# Autodesk Inventor assembly: electronicsLayout
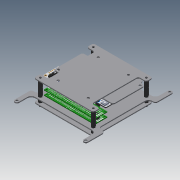
[picture p0: Inventor's stored thumbnail of the model, 180x180]
Saved by Autodesk Inventor 2018 (Build 220112000, 112)
## iProperties
Created: 2020-02-04
Part Number: electronicsLayout
Document SubType Name: Assembly
Designer: anirudh.bali
Author: anirudh.bali
## Documents named in this file (11)
- D:\Silicon Sharks\2019-2020\ElectronicsHousing\Prototype3\electronicsLayout.iam
- D:\Silicon Sharks\2019-2020\ElectronicsHousing\Prototype3\bottomPlate.ipt
- D:\Silicon Sharks\2019-2020\ElectronicsHousing\Components\standoffs\Separador plastico negro H-M M3x6x6mm.ipt
- D:\Silicon Sharks\2019-2020\ElectronicsHousing\Prototype3\groundPlate.ipt
- D:\Silicon Sharks\2019-2020\ElectronicsHousing\Components\Adafruit_BNO055_AP214.ipt
- D:\Silicon Sharks\2019-2020\ElectronicsHousing\Components\arduinoUnoDetailed.ipt
- D:\Silicon Sharks\2019-2020\ElectronicsHousing\Components\PCB2x8.ipt
- D:\Silicon Sharks\2019-2020\ElectronicsHousing\Prototype3\escPlate.ipt
- D:\Silicon Sharks\2019-2020\ElectronicsHousing\Components\standoffs\Separador plastico negro H-M M3x10x6mm.ipt
- D:\Silicon Sharks\2019-2020\ElectronicsHousing\Components\standoffs\Separador plastico negro H-M M3x12x6mm.ipt
- D:\Silicon Sharks\2019-2020\ElectronicsHousing\Prototype3\ethernetPlate.ipt
## Components (29 placed, 10 different names)
1. bottomPlate:1 — Mate:1, Mate:2, Mate:3, Mate:4, Mate:5, Mate:6, Mate:7, Mate:8
2. Separador plastico negro H-M M3x6x6mm:1 — Mate:1, Mate:5, Mate:10
3. Separador plastico negro H-M M3x6x6mm:2 — Mate:4, Mate:8, Mate:13
4. Separador plastico negro H-M M3x6x6mm:3 — Mate:3, Mate:7, Mate:9, Mate:12
5. Separador plastico negro H-M M3x6x6mm:4 — Mate:2, Mate:6, Mate:11
6. groundPlate:1 — Mate:9, Mate:10, Mate:11, Mate:12, Mate:13, Mate:14, Mate:15, Mate:16, Mate:17, Mate:18, Mate:19, Mate:20, Mate:21, Mate:25, Mate:26, Mate:27, Mate:28, Mate:29, Mate:54, Mate:55, Mate:56, Mate:57, Mate:58, Mate:59, Mate:60, Mate:61
7. Adafruit_BNO055_AP214:1 — Mate:25, Mate:26, Mate:27
8. arduinoUnoDetailed:1 — Mate:22, Mate:23, Mate:24, Mate:36, Mate:37, Mate:38, Mate:39, Mate:40, Mate:41
9. PCB2x8:1 — Mate:28, Mate:29, Mate:30, Mate:31, Mate:32, Mate:33
10. Separador plastico negro H-M M3x6x6mm:5 — Mate:16, Mate:17, Mate:22
11. Separador plastico negro H-M M3x6x6mm:6 — Mate:18, Mate:19, Mate:23
12. Separador plastico negro H-M M3x6x6mm:7 — Mate:20, Mate:21, Mate:24
13. Separador plastico negro H-M M3x6x6mm:8 — Mate:14, Mate:15
14. Separador plastico negro H-M M3x6x6mm:9 — Mate:30, Mate:33, Mate:34, Mate:35
15. Separador plastico negro H-M M3x6x6mm:10 — Mate:31, Mate:32
16. PCB2x8:2 — Mate:34, Mate:35
17. escPlate:1 — Mate:42, Mate:43, Mate:44, Mate:45
18. Separador plastico negro H-M M3x10x6mm:1 — Mate:40, Mate:41, Mate:45
19. Separador plastico negro H-M M3x10x6mm:2 — Mate:38, Mate:39, Mate:43
20. Separador plastico negro H-M M3x10x6mm:3 — Mate:36, Mate:37, Mate:42, Mate:44
21. Separador plastico negro H-M M3x12x6mm:1 — Mate:46, Mate:47, Mate:54, Flush:1
22. Separador plastico negro H-M M3x12x6mm:2 — Mate:52, Mate:53, Mate:60, Flush:4
23. Separador plastico negro H-M M3x12x6mm:3 — Mate:50, Mate:51, Mate:58, Flush:3
24. Separador plastico negro H-M M3x12x6mm:4 — Mate:48, Mate:49, Mate:56, Flush:2
25. Separador plastico negro H-M M3x12x6mm:5 — Mate:46, Mate:47, Mate:55, Flush:1, Mate:62, Mate:64
26. Separador plastico negro H-M M3x12x6mm:6 — Mate:52, Mate:53, Mate:61, Flush:4, Mate:65
27. Separador plastico negro H-M M3x12x6mm:7 — Mate:50, Mate:51, Mate:59, Flush:3, Mate:66
28. Separador plastico negro H-M M3x12x6mm:8 — Mate:48, Mate:49, Mate:57, Flush:2, Mate:63
29. ethernetPlate:1 — Mate:62, Mate:63, Mate:64, Mate:65, Mate:66
## Relationships (70: Mate 66, Flush 4)
- Mate:1: bottomPlate:1 ↔ Separador plastico negro H-M M3x6x6mm:1
- Mate:2: bottomPlate:1 ↔ Separador plastico negro H-M M3x6x6mm:4
- Mate:3: bottomPlate:1 ↔ Separador plastico negro H-M M3x6x6mm:3
- Mate:4: bottomPlate:1 ↔ Separador plastico negro H-M M3x6x6mm:2
- Mate:5: bottomPlate:1 ↔ Separador plastico negro H-M M3x6x6mm:1
- Mate:6: bottomPlate:1 ↔ Separador plastico negro H-M M3x6x6mm:4
- Mate:7: bottomPlate:1 ↔ Separador plastico negro H-M M3x6x6mm:3
- Mate:8: bottomPlate:1 ↔ Separador plastico negro H-M M3x6x6mm:2
- Mate:9: Separador plastico negro H-M M3x6x6mm:3 ↔ groundPlate:1
- Mate:10: Separador plastico negro H-M M3x6x6mm:1 ↔ groundPlate:1
- Mate:11: Separador plastico negro H-M M3x6x6mm:4 ↔ groundPlate:1
- Mate:12: Separador plastico negro H-M M3x6x6mm:3 ↔ groundPlate:1
- Mate:13: Separador plastico negro H-M M3x6x6mm:2 ↔ groundPlate:1
- Mate:14: groundPlate:1 ↔ Separador plastico negro H-M M3x6x6mm:8
- Mate:15: groundPlate:1 ↔ Separador plastico negro H-M M3x6x6mm:8
- Mate:16: groundPlate:1 ↔ Separador plastico negro H-M M3x6x6mm:5
- Mate:17: groundPlate:1 ↔ Separador plastico negro H-M M3x6x6mm:5
- Mate:18: groundPlate:1 ↔ Separador plastico negro H-M M3x6x6mm:6
- Mate:19: groundPlate:1 ↔ Separador plastico negro H-M M3x6x6mm:6
- Mate:20: groundPlate:1 ↔ Separador plastico negro H-M M3x6x6mm:7
- Mate:21: groundPlate:1 ↔ Separador plastico negro H-M M3x6x6mm:7
- Mate:22: arduinoUnoDetailed:1 ↔ Separador plastico negro H-M M3x6x6mm:5
- Mate:23: arduinoUnoDetailed:1 ↔ Separador plastico negro H-M M3x6x6mm:6
- Mate:24: arduinoUnoDetailed:1 ↔ Separador plastico negro H-M M3x6x6mm:7
- Mate:25: groundPlate:1 ↔ Adafruit_BNO055_AP214:1
- Mate:26: groundPlate:1 ↔ Adafruit_BNO055_AP214:1
- Mate:27: groundPlate:1 ↔ Adafruit_BNO055_AP214:1
- Mate:28: groundPlate:1 ↔ PCB2x8:1
- Mate:29: groundPlate:1 ↔ PCB2x8:1
- Mate:30: PCB2x8:1 ↔ Separador plastico negro H-M M3x6x6mm:9
- Mate:31: PCB2x8:1 ↔ Separador plastico negro H-M M3x6x6mm:10
- Mate:32: PCB2x8:1 ↔ Separador plastico negro H-M M3x6x6mm:10
- Mate:33: PCB2x8:1 ↔ Separador plastico negro H-M M3x6x6mm:9
- Mate:34: Separador plastico negro H-M M3x6x6mm:9 ↔ PCB2x8:2
- Mate:35: Separador plastico negro H-M M3x6x6mm:9 ↔ PCB2x8:2
- Mate:36: arduinoUnoDetailed:1 ↔ Separador plastico negro H-M M3x10x6mm:3
- Mate:37: arduinoUnoDetailed:1 ↔ Separador plastico negro H-M M3x10x6mm:3
- Mate:38: arduinoUnoDetailed:1 ↔ Separador plastico negro H-M M3x10x6mm:2
- Mate:39: arduinoUnoDetailed:1 ↔ Separador plastico negro H-M M3x10x6mm:2
- Mate:40: arduinoUnoDetailed:1 ↔ Separador plastico negro H-M M3x10x6mm:1
- Mate:41: arduinoUnoDetailed:1 ↔ Separador plastico negro H-M M3x10x6mm:1
- Mate:42: escPlate:1 ↔ Separador plastico negro H-M M3x10x6mm:3
- Mate:43: escPlate:1 ↔ Separador plastico negro H-M M3x10x6mm:2
- Mate:44: escPlate:1 ↔ Separador plastico negro H-M M3x10x6mm:3
- Mate:45: escPlate:1 ↔ Separador plastico negro H-M M3x10x6mm:1
- Mate:46: Separador plastico negro H-M M3x12x6mm:1 ↔ Separador plastico negro H-M M3x12x6mm:5
- Mate:47: Separador plastico negro H-M M3x12x6mm:1 ↔ Separador plastico negro H-M M3x12x6mm:5
- Mate:48: Separador plastico negro H-M M3x12x6mm:4 ↔ Separador plastico negro H-M M3x12x6mm:8
- Mate:49: Separador plastico negro H-M M3x12x6mm:4 ↔ Separador plastico negro H-M M3x12x6mm:8
- Mate:50: Separador plastico negro H-M M3x12x6mm:3 ↔ Separador plastico negro H-M M3x12x6mm:7
- Mate:51: Separador plastico negro H-M M3x12x6mm:3 ↔ Separador plastico negro H-M M3x12x6mm:7
- Mate:52: Separador plastico negro H-M M3x12x6mm:2 ↔ Separador plastico negro H-M M3x12x6mm:6
- Mate:53: Separador plastico negro H-M M3x12x6mm:2 ↔ Separador plastico negro H-M M3x12x6mm:6
- Mate:54: groundPlate:1 ↔ Separador plastico negro H-M M3x12x6mm:1
- Mate:55: groundPlate:1 ↔ Separador plastico negro H-M M3x12x6mm:5
- Flush:1: Separador plastico negro H-M M3x12x6mm:1 ↔ Separador plastico negro H-M M3x12x6mm:5
- Mate:56: groundPlate:1 ↔ Separador plastico negro H-M M3x12x6mm:4
- Mate:57: groundPlate:1 ↔ Separador plastico negro H-M M3x12x6mm:8
- Flush:2: Separador plastico negro H-M M3x12x6mm:4 ↔ Separador plastico negro H-M M3x12x6mm:8
- Mate:58: groundPlate:1 ↔ Separador plastico negro H-M M3x12x6mm:3
- Mate:59: groundPlate:1 ↔ Separador plastico negro H-M M3x12x6mm:7
- Flush:3: Separador plastico negro H-M M3x12x6mm:3 ↔ Separador plastico negro H-M M3x12x6mm:7
- Mate:60: groundPlate:1 ↔ Separador plastico negro H-M M3x12x6mm:2
- Mate:61: groundPlate:1 ↔ Separador plastico negro H-M M3x12x6mm:6
- Flush:4: Separador plastico negro H-M M3x12x6mm:2 ↔ Separador plastico negro H-M M3x12x6mm:6
- Mate:62: Separador plastico negro H-M M3x12x6mm:5 ↔ ethernetPlate:1
- Mate:63: Separador plastico negro H-M M3x12x6mm:8 ↔ ethernetPlate:1
- Mate:64: Separador plastico negro H-M M3x12x6mm:5 ↔ ethernetPlate:1
- Mate:65: Separador plastico negro H-M M3x12x6mm:6 ↔ ethernetPlate:1
- Mate:66: Separador plastico negro H-M M3x12x6mm:7 ↔ ethernetPlate:1
